# Autodesk Inventor assembly: BallBot_macro
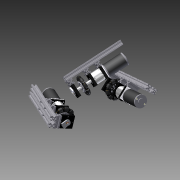
[picture p0: Inventor's stored thumbnail of the model, 180x180]
Saved by Autodesk Inventor 2012 (Build 160160000, 160)
## iProperties
Created: 2012-10-25
Part Number: BallBot_macro
Document SubType Name: Assembly
Designer: Andrew G. Meyer
Author: Andrew G. Meyer
## Documents named in this file (2)
- C:\Users\Andrew G. Meyer\Documents\Projects\BallBot\macro\CAD\BallBot_macro.iam
- C:\Users\Andrew G. Meyer\Documents\Projects\BallBot\macro\CAD\Drivetrain_Module.iam
## Components (3 placed, 1 different names)
1. Drivetrain_Module:1 [sub-assembly] — Angle:1, Angle:2
2. Drivetrain_Module:2 [sub-assembly] — Angle:1, Angle:3
3. Drivetrain_Module:3 [sub-assembly] — Angle:2, Angle:3
## Relationships (3: Angle 3)
- Angle:1 (120 deg): Drivetrain_Module:1 ↔ Drivetrain_Module:2
- Angle:2 (120 deg): Drivetrain_Module:1 ↔ Drivetrain_Module:3
- Angle:3 (120 deg): Drivetrain_Module:2 ↔ Drivetrain_Module:3
